# Autodesk Inventor assembly: OpenROV_Dev_Assy
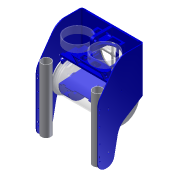
[picture p0: Inventor's stored thumbnail of the model, 180x180]
Saved by Autodesk Inventor 2012 (Build 160160000, 160)
## iProperties
Created: 2012-07-04
Part Number: OpenROV_Dev_Assy
Document SubType Name: Assembly
Designer: user
Author: user
## Documents named in this file (18)
- C:\Users\user\Desktop\CLEAN ME\OpenROV\openrov-hardware\OpenROV 2.3.2 Dev\OpenROV_Dev_Assy.iam
- C:\Users\user\Desktop\CLEAN ME\OpenROV\openrov-hardware\OpenROV 2.3.2 Dev\OpenROV_Dev_Bulkhead.ipt
- C:\Users\user\Desktop\CLEAN ME\OpenROV\openrov-hardware\OpenROV 2.3.2 Dev\OpenROV_Dev_Shroud_Brace_Mount.ipt
- C:\Users\user\Desktop\CLEAN ME\OpenROV\openrov-hardware\OpenROV 2.3.2 Dev\OpenROV_Dev_Vertical_Motor_Mount.ipt
- C:\Users\user\Desktop\CLEAN ME\OpenROV\openrov-hardware\OpenROV 2.3.2 Dev\OpenROV_Dev_Horizontal_Motor_Mount.ipt
- C:\Users\user\Desktop\CLEAN ME\OpenROV\openrov-hardware\OpenROV 2.3.2 Dev\OpenROV_Dev_Electronics_Tube_Brace.ipt
- C:\Users\user\Desktop\CLEAN ME\OpenROV\openrov-hardware\OpenROV 2.3.2 Dev\OpenROV_Dev_Shroud_Brace.ipt
- C:\Users\user\Desktop\CLEAN ME\OpenROV\openrov-hardware\OpenROV 2.3.2 Dev\OpenROV_Dev_Handle.ipt
- C:\Users\user\Desktop\CLEAN ME\OpenROV\openrov-hardware\OpenROV 2.3.2 Dev\OpenROV_Dev_Top_Plate.ipt
- C:\Users\user\Desktop\CLEAN ME\OpenROV\openrov-hardware\OpenROV 2.3.2 Dev\OpenROV_Dev_Bulkhead_Brace.ipt
- C:\Users\user\Desktop\CLEAN ME\OpenROV\openrov-hardware\OpenROV 2.3.2 Dev\OpenROV_Dev_Shell.ipt
- C:\Users\user\Desktop\CLEAN ME\OpenROV\openrov-hardware\OpenROV 2.3.2 Dev\OpenROV_Dev_Vertical_Thruster_Guard.ipt
- C:\Users\user\Desktop\CLEAN ME\OpenROV\openrov-hardware\OpenROV 2.3.2 Dev\OpenROV_Dev_Electronics_Tube.ipt
- C:\Users\user\Desktop\CLEAN ME\OpenROV\openrov-hardware\OpenROV 2.3.2 Dev\OpenROV_Dev_EChassis.iam
- C:\Users\user\Desktop\CLEAN ME\OpenROV\openrov-hardware\OpenROV 2.3.2 Dev\OpenROV_Dev_Port_EndCap.iam
- C:\Users\user\Desktop\CLEAN ME\OpenROV\openrov-hardware\OpenROV 2.3.2 Dev\OpenROV_Dev_Starbord_EndCap.iam
- C:\Users\user\Desktop\CLEAN ME\OpenROV\openrov-hardware\OpenROV 2.3.2 Dev\OpenROV_Dev_Prop_Shroud.ipt
- C:\Users\user\Desktop\CLEAN ME\OpenROV\openrov-hardware\OpenROV 2.3.2 Dev\OpenROV_Dev_Battery_Tube.ipt
## Components (26 placed, 17 different names)
1. OpenROV_Dev_Bulkhead:1 — Mate:7, Mate:8, Mate:9, Mate:15, Mate:16, Flush:5, Mate:17, Mate:18, Flush:6, Mate:27, Mate:30, Flush:12, Mate:33
2. OpenROV_Dev_Shroud_Brace_Mount:1 — Mate:1, Mate:2, Mate:3, Mate:9, Mate:12, Mate:31, Mate:47
3. OpenROV_Dev_Shroud_Brace_Mount:2 — Mate:4, Mate:5, Mate:6, Mate:8, Mate:19, Mate:20, Mate:21, Mate:48
4. OpenROV_Dev_Vertical_Motor_Mount:1 — Mate:1, Mate:2, Mate:3, Mate:4, Mate:5, Mate:6, Mate:7, Mate:10, Mate:11
5. OpenROV_Dev_Horizontal_Motor_Mount:1 — Mate:10, Mate:11, Mate:12
6. OpenROV_Dev_Electronics_Tube_Brace:1 — Mate:14, Flush:3, Flush:4, Mate:18, Flush:6, Mate:28, Mate:29
7. OpenROV_Dev_Electronics_Tube_Brace:2 — Mate:14, Flush:3, Flush:4, Mate:17, Mate:36, Mate:43
8. OpenROV_Dev_Electronics_Tube_Brace:3 — Mate:13, Flush:1, Flush:2, Mate:15, Mate:16
9. OpenROV_Dev_Electronics_Tube_Brace:4 — Mate:13, Flush:1, Flush:2, Flush:5
10. OpenROV_Dev_Shroud_Brace:1 — Mate:19, Mate:20, Mate:21, Mate:24, Mate:25, Mate:26, Mate:45, Mate:46
11. OpenROV_Dev_Handle:1 — Mate:22, Flush:7, Flush:8, Flush:11
12. OpenROV_Dev_Handle:2 — Mate:22, Flush:7, Mate:23, Flush:8, Flush:9, Flush:10, Flush:11, Mate:24, Mate:25
13. OpenROV_Dev_Handle:3 — Mate:23, Flush:9, Flush:10, Mate:26
14. OpenROV_Dev_Top_Plate:1 — Mate:27, Mate:28, Mate:29, Mate:32, Flush:13, Mate:34, Mate:49, Mate:50
15. OpenROV_Dev_Bulkhead_Brace:1 — Mate:30, Mate:31, Flush:12
16. OpenROV_Dev_Shell:1 — Mate:32, Mate:33, Flush:13, Mate:35
17. OpenROV_Dev_Vertical_Thruster_Guard:1 — Mate:34, Mate:35
18. OpenROV_Dev_Electronics_Tube:1 — Mate:36, Mate:37, Mate:38, Mate:39, Mate:40, Mate:41, Mate:42
19. OpenROV_Dev_EChassis:1 [sub-assembly] — Mate:37, Mate:38, Mate:44
20. OpenROV_Dev_Port_EndCap:1 [sub-assembly] — Mate:39, Mate:40, Mate:43, Mate:44
21. OpenROV_Dev_Starbord_EndCap:1 [sub-assembly] — Mate:41, Mate:42
22. OpenROV_Dev_Prop_Shroud:1 — Mate:45, Mate:47
23. OpenROV_Dev_Prop_Shroud:2 — Mate:46, Mate:48
24. OpenROV_Dev_Prop_Shroud:3 — Mate:49, Mate:50
25. OpenROV_Dev_Battery_Tube:1
26. OpenROV_Dev_Battery_Tube:2
## Relationships (63: Mate 50, Flush 13)
- Mate:1: OpenROV_Dev_Shroud_Brace_Mount:1 ↔ OpenROV_Dev_Vertical_Motor_Mount:1
- Mate:2: OpenROV_Dev_Shroud_Brace_Mount:1 ↔ OpenROV_Dev_Vertical_Motor_Mount:1
- Mate:3: OpenROV_Dev_Shroud_Brace_Mount:1 ↔ OpenROV_Dev_Vertical_Motor_Mount:1
- Mate:4: OpenROV_Dev_Shroud_Brace_Mount:2 ↔ OpenROV_Dev_Vertical_Motor_Mount:1
- Mate:5: OpenROV_Dev_Shroud_Brace_Mount:2 ↔ OpenROV_Dev_Vertical_Motor_Mount:1
- Mate:6: OpenROV_Dev_Shroud_Brace_Mount:2 ↔ OpenROV_Dev_Vertical_Motor_Mount:1
- Mate:7: OpenROV_Dev_Bulkhead:1 ↔ OpenROV_Dev_Vertical_Motor_Mount:1
- Mate:8: OpenROV_Dev_Bulkhead:1 ↔ OpenROV_Dev_Shroud_Brace_Mount:2
- Mate:9: OpenROV_Dev_Bulkhead:1 ↔ OpenROV_Dev_Shroud_Brace_Mount:1
- Mate:10: OpenROV_Dev_Vertical_Motor_Mount:1 ↔ OpenROV_Dev_Horizontal_Motor_Mount:1
- Mate:11: OpenROV_Dev_Vertical_Motor_Mount:1 ↔ OpenROV_Dev_Horizontal_Motor_Mount:1
- Mate:12: OpenROV_Dev_Shroud_Brace_Mount:1 ↔ OpenROV_Dev_Horizontal_Motor_Mount:1
- Mate:13: OpenROV_Dev_Electronics_Tube_Brace:3 ↔ OpenROV_Dev_Electronics_Tube_Brace:4
- Flush:1: OpenROV_Dev_Electronics_Tube_Brace:3 ↔ OpenROV_Dev_Electronics_Tube_Brace:4
- Flush:2: OpenROV_Dev_Electronics_Tube_Brace:3 ↔ OpenROV_Dev_Electronics_Tube_Brace:4
- Mate:14: OpenROV_Dev_Electronics_Tube_Brace:1 ↔ OpenROV_Dev_Electronics_Tube_Brace:2
- Flush:3: OpenROV_Dev_Electronics_Tube_Brace:1 ↔ OpenROV_Dev_Electronics_Tube_Brace:2
- Flush:4: OpenROV_Dev_Electronics_Tube_Brace:1 ↔ OpenROV_Dev_Electronics_Tube_Brace:2
- Mate:15: OpenROV_Dev_Bulkhead:1 ↔ OpenROV_Dev_Electronics_Tube_Brace:3
- Mate:16: OpenROV_Dev_Bulkhead:1 ↔ OpenROV_Dev_Electronics_Tube_Brace:3
- Flush:5: OpenROV_Dev_Bulkhead:1 ↔ OpenROV_Dev_Electronics_Tube_Brace:4
- Mate:17: OpenROV_Dev_Bulkhead:1 ↔ OpenROV_Dev_Electronics_Tube_Brace:2
- Mate:18: OpenROV_Dev_Bulkhead:1 ↔ OpenROV_Dev_Electronics_Tube_Brace:1
- Flush:6: OpenROV_Dev_Bulkhead:1 ↔ OpenROV_Dev_Electronics_Tube_Brace:1
- Mate:19: OpenROV_Dev_Shroud_Brace_Mount:2 ↔ OpenROV_Dev_Shroud_Brace:1
- Mate:20: OpenROV_Dev_Shroud_Brace_Mount:2 ↔ OpenROV_Dev_Shroud_Brace:1
- Mate:21: OpenROV_Dev_Shroud_Brace_Mount:2 ↔ OpenROV_Dev_Shroud_Brace:1
- Mate:22: OpenROV_Dev_Handle:1 ↔ OpenROV_Dev_Handle:2
- Flush:7: OpenROV_Dev_Handle:1 ↔ OpenROV_Dev_Handle:2
- Mate:23: OpenROV_Dev_Handle:2 ↔ OpenROV_Dev_Handle:3
- Flush:8: OpenROV_Dev_Handle:1 ↔ OpenROV_Dev_Handle:2
- Flush:9: OpenROV_Dev_Handle:2 ↔ OpenROV_Dev_Handle:3
- Flush:10: OpenROV_Dev_Handle:2 ↔ OpenROV_Dev_Handle:3
- Flush:11: OpenROV_Dev_Handle:1 ↔ OpenROV_Dev_Handle:2
- Mate:24: OpenROV_Dev_Shroud_Brace:1 ↔ OpenROV_Dev_Handle:2
- Mate:25: OpenROV_Dev_Shroud_Brace:1 ↔ OpenROV_Dev_Handle:2
- Mate:26: OpenROV_Dev_Shroud_Brace:1 ↔ OpenROV_Dev_Handle:3
- Mate:27: OpenROV_Dev_Bulkhead:1 ↔ OpenROV_Dev_Top_Plate:1
- Mate:28: OpenROV_Dev_Electronics_Tube_Brace:1 ↔ OpenROV_Dev_Top_Plate:1
- Mate:29: OpenROV_Dev_Electronics_Tube_Brace:1 ↔ OpenROV_Dev_Top_Plate:1
- Mate:30: OpenROV_Dev_Bulkhead:1 ↔ OpenROV_Dev_Bulkhead_Brace:1
- Mate:31: OpenROV_Dev_Shroud_Brace_Mount:1 ↔ OpenROV_Dev_Bulkhead_Brace:1
- Flush:12: OpenROV_Dev_Bulkhead:1 ↔ OpenROV_Dev_Bulkhead_Brace:1
- Mate:32: OpenROV_Dev_Top_Plate:1 ↔ OpenROV_Dev_Shell:1
- Mate:33: OpenROV_Dev_Bulkhead:1 ↔ OpenROV_Dev_Shell:1
- Flush:13: OpenROV_Dev_Top_Plate:1 ↔ OpenROV_Dev_Shell:1
- Mate:34: OpenROV_Dev_Top_Plate:1 ↔ OpenROV_Dev_Vertical_Thruster_Guard:1
- Mate:35: OpenROV_Dev_Shell:1 ↔ OpenROV_Dev_Vertical_Thruster_Guard:1
- Mate:36: OpenROV_Dev_Electronics_Tube_Brace:2 ↔ OpenROV_Dev_Electronics_Tube:1
- Mate:37: OpenROV_Dev_Electronics_Tube:1 ↔ OpenROV_Dev_EChassis:1
- Mate:38: OpenROV_Dev_Electronics_Tube:1 ↔ OpenROV_Dev_EChassis:1
- Mate:39: OpenROV_Dev_Electronics_Tube:1 ↔ OpenROV_Dev_Port_EndCap:1
- Mate:40: OpenROV_Dev_Electronics_Tube:1 ↔ OpenROV_Dev_Port_EndCap:1
- Mate:41: OpenROV_Dev_Electronics_Tube:1 ↔ OpenROV_Dev_Starbord_EndCap:1
- Mate:42: OpenROV_Dev_Electronics_Tube:1 ↔ OpenROV_Dev_Starbord_EndCap:1
- Mate:43: OpenROV_Dev_Electronics_Tube_Brace:2 ↔ OpenROV_Dev_Port_EndCap:1
- Mate:44: OpenROV_Dev_EChassis:1 ↔ OpenROV_Dev_Port_EndCap:1
- Mate:45: OpenROV_Dev_Shroud_Brace:1 ↔ OpenROV_Dev_Prop_Shroud:1
- Mate:46: OpenROV_Dev_Shroud_Brace:1 ↔ OpenROV_Dev_Prop_Shroud:2
- Mate:47: OpenROV_Dev_Shroud_Brace_Mount:1 ↔ OpenROV_Dev_Prop_Shroud:1
- Mate:48: OpenROV_Dev_Shroud_Brace_Mount:2 ↔ OpenROV_Dev_Prop_Shroud:2
- Mate:49: OpenROV_Dev_Top_Plate:1 ↔ OpenROV_Dev_Prop_Shroud:3
- Mate:50: OpenROV_Dev_Top_Plate:1 ↔ OpenROV_Dev_Prop_Shroud:3
